# Autodesk Inventor assembly: EnsemblePCB
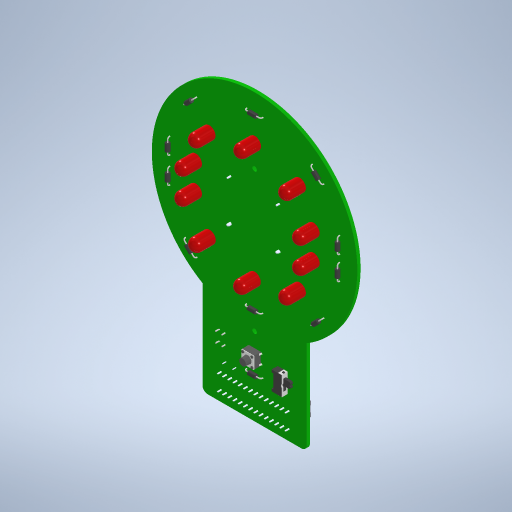
[picture p0: Inventor's stored thumbnail of the model, 512x512]
Saved by Autodesk Inventor 2024 (Build 280153000, 153)
## iProperties
Created: 2023-11-16
Part Number: EnsemblePCB
Document SubType Name: Assembly
Designer: digiacom
Author: digiacom
## Documents named in this file (11)
- D:\Projet\Perso\ATMegaSpin\Inventor\EnsemblePCB.iam
- D:\Projet\Perso\ATMegaSpin\3DModel\ATMegaSpin\ATMegaSpin.ipt
- D:\Projet\Perso\ATMegaSpin\3DModel\Parts\BS-7--3DModel-STEP-1\BS-7--3DModel-STEP-1.ipt
- D:\Projet\Perso\ATMegaSpin\3DModel\Parts\ED281DT\ED281DT.ipt
- D:\Projet\Perso\ATMegaSpin\3DModel\Parts\ATMEGA328P-PU\ATMEGA328P-PU.ipt
- D:\Projet\Perso\ATMegaSpin\3DModel\Parts\ECS-160-18-4X-CKM\ECS-160-18-4X-CKM.ipt
- D:\Projet\Perso\ATMegaSpin\3DModel\Parts\CAP_K-SERIES_15-L2_VIS\CAP_K-SERIES_15-L2_VIS.ipt
- D:\Projet\Perso\ATMegaSpin\3DModel\Parts\STA_CF18_STP\STA_CF18_STP.ipt
- D:\Projet\Perso\ATMegaSpin\3DModel\Parts\LED_HLMP-47XX_BRA\LED_HLMP-47XX_BRA.ipt
- D:\Projet\Perso\ATMegaSpin\3DModel\Parts\CUI_DEVICES_TS02-66-60-BK-160-SCR-D\CUI_DEVICES_TS02-66-60-BK-160-SCR-D.ipt
- D:\Projet\Perso\ATMegaSpin\3DModel\Parts\MFS101D-6-Z\MFS101D-6-Z.ipt
## Components (31 placed, 10 different names)
1. ATMegaSpin:1 — Placage:2, Placage:3, Placage:4, Placage:5, Placage:6, Placage:7, Placage:9, Placage:10, Placage:11, Placage:12, Placage:13, Placage:14, Placage:15, Placage:16, Placage:17, Placage:18, Placage:19, Placage:20, Placage:21, Placage:22, Placage:23, Placage:24, Placage:25, Placage:26, Placage:27, Placage:28, Placage:29, Placage:30, Placage:31, Placage:32, Placage:33, Placage:34, Placage:35, Placage:36, Placage:37, Placage:38, Placage:39, Placage:40, Placage:41, Placage:42, Placage:43, Placage:44, Placage:45, Placage:46, Placage:47, Placage:48, Placage:49, Placage:50, Placage:51, Placage:52, Placage:53, Placage:54, Placage:55, Placage:56, Placage:57, Placage:58, Placage:59, Placage:60, Placage:61, Placage:62, Placage:63, Placage:64, Placage:65, Placage:66, Placage:67, Placage:68, Placage:69, Placage:70, Placage:71
2. BS-7--3DModel-STEP-1:1 — Placage:2, Placage:3
3. BS-7--3DModel-STEP-1:2 — Placage:4, Placage:5
4. ED281DT:2
5. ATMEGA328P-PU:1
6. ECS-160-18-4X-CKM:1 — Placage:6, Placage:7
7. CAP_K-SERIES_15-L2_VIS:1 — Placage:10
8. CAP_K-SERIES_15-L2_VIS:2 — Placage:9
9. STA_CF18_STP:1 — Placage:13, Placage:14
10. STA_CF18_STP:2 — Placage:15, Placage:16, Placage:17
11. STA_CF18_STP:3 — Placage:18, Placage:19
12. STA_CF18_STP:4 — Placage:20, Placage:21, Placage:22
13. STA_CF18_STP:5 — Placage:23, Placage:24, Placage:25
14. STA_CF18_STP:6 — Placage:26, Placage:27, Placage:28
15. STA_CF18_STP:7 — Placage:29, Placage:30, Placage:31
16. STA_CF18_STP:8 — Placage:32, Placage:33, Placage:34
17. STA_CF18_STP:9 — Placage:35, Placage:36, Placage:37
18. STA_CF18_STP:10 — Placage:11, Placage:12
19. STA_CF18_STP:11 — Placage:38, Placage:39, Placage:40
20. LED_HLMP-47XX_BRA:1 — Placage:59, Placage:60, Placage:61
21. LED_HLMP-47XX_BRA:2 — Placage:58, Placage:62, Placage:63
22. LED_HLMP-47XX_BRA:3 — Placage:57, Placage:64, Placage:65
23. LED_HLMP-47XX_BRA:4 — Placage:56, Placage:66, Placage:67
24. LED_HLMP-47XX_BRA:5 — Placage:55, Placage:68
25. LED_HLMP-47XX_BRA:6 — Placage:53, Placage:54
26. LED_HLMP-47XX_BRA:7 — Placage:50, Placage:51, Placage:52
27. LED_HLMP-47XX_BRA:8 — Placage:44, Placage:45, Placage:46
28. LED_HLMP-47XX_BRA:9 — Placage:41, Placage:42, Placage:43
29. LED_HLMP-47XX_BRA:10 — Placage:47, Placage:48, Placage:49
30. CUI_DEVICES_TS02-66-60-BK-160-SCR-D:1 — Placage:69
31. MFS101D-6-Z:1 — Placage:70, Placage:71
## Relationships (69: Mate 69)
- Placage:2 [Mate]: ATMegaSpin:1 ↔ BS-7--3DModel-STEP-1:1
- Placage:3 [Mate] (0.7 mm): ATMegaSpin:1 ↔ BS-7--3DModel-STEP-1:1
- Placage:4 [Mate]: ATMegaSpin:1 ↔ BS-7--3DModel-STEP-1:2
- Placage:5 [Mate] (-0.35 mm): ATMegaSpin:1 ↔ BS-7--3DModel-STEP-1:2
- Placage:6 [Mate]: ATMegaSpin:1 ↔ ECS-160-18-4X-CKM:1
- Placage:7 [Mate]: ATMegaSpin:1 ↔ ECS-160-18-4X-CKM:1
- Placage:9 [Mate]: ATMegaSpin:1 ↔ CAP_K-SERIES_15-L2_VIS:2
- Placage:10 [Mate]: ATMegaSpin:1 ↔ CAP_K-SERIES_15-L2_VIS:1
- Placage:11 [Mate]: ATMegaSpin:1 ↔ STA_CF18_STP:10
- Placage:12 [Mate] (1 mm): ATMegaSpin:1 ↔ STA_CF18_STP:10
- Placage:13 [Mate] (1 mm): ATMegaSpin:1 ↔ STA_CF18_STP:1
- Placage:14 [Mate]: ATMegaSpin:1 ↔ STA_CF18_STP:1
- Placage:15 [Mate] (1 mm): ATMegaSpin:1 ↔ STA_CF18_STP:2
- Placage:16 [Mate]: ATMegaSpin:1 ↔ STA_CF18_STP:2
- Placage:17 [Mate]: ATMegaSpin:1 ↔ STA_CF18_STP:2
- Placage:18 [Mate] (1 mm): ATMegaSpin:1 ↔ STA_CF18_STP:3
- Placage:19 [Mate]: ATMegaSpin:1 ↔ STA_CF18_STP:3
- Placage:20 [Mate] (1 mm): ATMegaSpin:1 ↔ STA_CF18_STP:4
- Placage:21 [Mate]: ATMegaSpin:1 ↔ STA_CF18_STP:4
- Placage:22 [Mate]: ATMegaSpin:1 ↔ STA_CF18_STP:4
- Placage:23 [Mate] (1 mm): ATMegaSpin:1 ↔ STA_CF18_STP:5
- Placage:24 [Mate]: ATMegaSpin:1 ↔ STA_CF18_STP:5
- Placage:25 [Mate]: ATMegaSpin:1 ↔ STA_CF18_STP:5
- Placage:26 [Mate] (1 mm): ATMegaSpin:1 ↔ STA_CF18_STP:6
- Placage:27 [Mate]: ATMegaSpin:1 ↔ STA_CF18_STP:6
- Placage:28 [Mate]: ATMegaSpin:1 ↔ STA_CF18_STP:6
- Placage:29 [Mate] (1 mm): ATMegaSpin:1 ↔ STA_CF18_STP:7
- Placage:30 [Mate]: ATMegaSpin:1 ↔ STA_CF18_STP:7
- Placage:31 [Mate]: ATMegaSpin:1 ↔ STA_CF18_STP:7
- Placage:32 [Mate] (1 mm): ATMegaSpin:1 ↔ STA_CF18_STP:8
- Placage:33 [Mate]: ATMegaSpin:1 ↔ STA_CF18_STP:8
- Placage:34 [Mate]: ATMegaSpin:1 ↔ STA_CF18_STP:8
- Placage:35 [Mate] (1 mm): ATMegaSpin:1 ↔ STA_CF18_STP:9
- Placage:36 [Mate]: ATMegaSpin:1 ↔ STA_CF18_STP:9
- Placage:37 [Mate]: ATMegaSpin:1 ↔ STA_CF18_STP:9
- Placage:38 [Mate] (1 mm): ATMegaSpin:1 ↔ STA_CF18_STP:11
- Placage:39 [Mate]: ATMegaSpin:1 ↔ STA_CF18_STP:11
- Placage:40 [Mate]: ATMegaSpin:1 ↔ STA_CF18_STP:11
- Placage:41 [Mate]: ATMegaSpin:1 ↔ LED_HLMP-47XX_BRA:9
- Placage:42 [Mate]: ATMegaSpin:1 ↔ LED_HLMP-47XX_BRA:9
- Placage:43 [Mate]: ATMegaSpin:1 ↔ LED_HLMP-47XX_BRA:9
- Placage:44 [Mate]: ATMegaSpin:1 ↔ LED_HLMP-47XX_BRA:8
- Placage:45 [Mate]: ATMegaSpin:1 ↔ LED_HLMP-47XX_BRA:8
- Placage:46 [Mate]: ATMegaSpin:1 ↔ LED_HLMP-47XX_BRA:8
- Placage:47 [Mate]: ATMegaSpin:1 ↔ LED_HLMP-47XX_BRA:10
- Placage:48 [Mate]: ATMegaSpin:1 ↔ LED_HLMP-47XX_BRA:10
- Placage:49 [Mate]: ATMegaSpin:1 ↔ LED_HLMP-47XX_BRA:10
- Placage:50 [Mate]: ATMegaSpin:1 ↔ LED_HLMP-47XX_BRA:7
- Placage:51 [Mate]: ATMegaSpin:1 ↔ LED_HLMP-47XX_BRA:7
- Placage:52 [Mate]: ATMegaSpin:1 ↔ LED_HLMP-47XX_BRA:7
- Placage:53 [Mate]: ATMegaSpin:1 ↔ LED_HLMP-47XX_BRA:6
- Placage:54 [Mate]: ATMegaSpin:1 ↔ LED_HLMP-47XX_BRA:6
- Placage:55 [Mate]: ATMegaSpin:1 ↔ LED_HLMP-47XX_BRA:5
- Placage:56 [Mate]: ATMegaSpin:1 ↔ LED_HLMP-47XX_BRA:4
- Placage:57 [Mate]: ATMegaSpin:1 ↔ LED_HLMP-47XX_BRA:3
- Placage:58 [Mate]: ATMegaSpin:1 ↔ LED_HLMP-47XX_BRA:2
- Placage:59 [Mate]: ATMegaSpin:1 ↔ LED_HLMP-47XX_BRA:1
- Placage:60 [Mate]: ATMegaSpin:1 ↔ LED_HLMP-47XX_BRA:1
- Placage:61 [Mate]: ATMegaSpin:1 ↔ LED_HLMP-47XX_BRA:1
- Placage:62 [Mate]: ATMegaSpin:1 ↔ LED_HLMP-47XX_BRA:2
- Placage:63 [Mate]: ATMegaSpin:1 ↔ LED_HLMP-47XX_BRA:2
- Placage:64 [Mate]: ATMegaSpin:1 ↔ LED_HLMP-47XX_BRA:3
- Placage:65 [Mate]: ATMegaSpin:1 ↔ LED_HLMP-47XX_BRA:3
- Placage:66 [Mate]: ATMegaSpin:1 ↔ LED_HLMP-47XX_BRA:4
- Placage:67 [Mate]: ATMegaSpin:1 ↔ LED_HLMP-47XX_BRA:4
- Placage:68 [Mate]: ATMegaSpin:1 ↔ LED_HLMP-47XX_BRA:5
- Placage:69 [Mate]: ATMegaSpin:1 ↔ CUI_DEVICES_TS02-66-60-BK-160-SCR-D:1
- Placage:70 [Mate]: ATMegaSpin:1 ↔ MFS101D-6-Z:1
- Placage:71 [Mate]: ATMegaSpin:1 ↔ MFS101D-6-Z:1
